# Autodesk Inventor assembly: tela
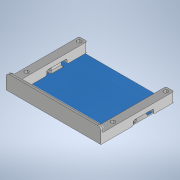
[picture p0: Inventor's stored thumbnail of the model, 180x180]
Saved by Autodesk Inventor 2020 (Build 240168000, 168)
## iProperties
Created: 2019-09-20
Part Number: tela
Document SubType Name: Assembly
Designer: Acer
Author: Acer
## Documents named in this file (3)
- C:\Users\Acer\Documents\Autinho\tela.iam
- C:\Users\Acer\Documents\Autinho\SuporteTelaLed.ipt
- C:\Users\Acer\Documents\Autinho\Tela Led.ipt
## Components (2 placed, 2 different names)
1. SuporteTelaLed:1 — Mate:1, Mate:2, Mate:3
2. Tela Led:1 — Mate:1, Mate:2, Mate:3
## Relationships (3: Mate 3)
- Mate:1: SuporteTelaLed:1 ↔ Tela Led:1
- Mate:2: SuporteTelaLed:1 ↔ Tela Led:1
- Mate:3: SuporteTelaLed:1 ↔ Tela Led:1
